# Autodesk Inventor assembly: sensorBoard
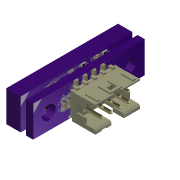
[picture p0: Inventor's stored thumbnail of the model, 180x180]
Saved by Autodesk Inventor 2017 (Build 210142000, 142)
## iProperties
Created: 2016-02-15
Part Number: sensorBoard
Document SubType Name: Assembly
Designer: sawai
Author: sawai
## Documents named in this file (4)
- C:\Users\sawaiz\oneDrive\projects\mppcSensor\cad\mppcSensor.iam
- C:\Users\sawaiz\oneDrive\projects\mppcSensor\cad\sensorBoardB\boardB.iam
- C:\Users\sawaiz\oneDrive\projects\mppcSensor\cad\sensorBoardC\boardC.iam
- C:\Users\sawaiz\oneDrive\projects\mppcSensor\cad\sensorBoardA\boardA.ipt
## Components (3 placed, 3 different names)
1. boardC:1 [sub-assembly] — Mate:1, Flush:2, Flush:4
2. boardB:1 [sub-assembly] — Mate:1, Mate:2, Flush:1, Flush:2, Flush:3, Flush:4
3. boardA:1 — Mate:2, Flush:1, Flush:3
## Relationships (6: Flush 4, Mate 2)
- Mate:1: boardC:1 ↔ boardB:1
- Mate:2: boardB:1 ↔ boardA:1
- Flush:1: boardB:1 ↔ boardA:1
- Flush:2: boardC:1 ↔ boardB:1
- Flush:3: boardB:1 ↔ boardA:1
- Flush:4: boardC:1 ↔ boardB:1
